# Autodesk Inventor assembly: motor
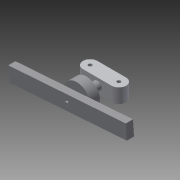
[picture p0: Inventor's stored thumbnail of the model, 180x180]
Saved by Autodesk Inventor 2013 (Build 170138000, 138)
## iProperties
Created: 2013-01-16
Part Number: motor
Document SubType Name: Assembly
Designer: geohot
Author: geohot
## Documents named in this file (5)
- C:\Users\geohot\Documents\GitHub\quadrotor\cad\motor.iam
- C:\Users\geohot\Documents\GitHub\quadrotor\cad\can.ipt
- C:\Users\geohot\Documents\GitHub\quadrotor\cad\stator.ipt
- C:\Users\geohot\Documents\GitHub\quadrotor\cad\prop.ipt
- C:\Users\geohot\Documents\GitHub\quadrotor\cad\motormount.ipt
## Components (4 placed, 4 different names)
1. can:1 — Insert:1, Insert:2
2. stator:1 — Insert:1, Flush:1
3. prop:1 — Insert:2
4. motormount:1 — Flush:1
## Relationships (3: Insert 2, Flush 1)
- Insert:1 (-2.2 mm): can:1 ↔ stator:1
- Insert:2 (1.524 mm): can:1 ↔ prop:1
- Flush:1: stator:1 ↔ motormount:1
